# Autodesk Inventor assembly: ParticleLauncherwCollector
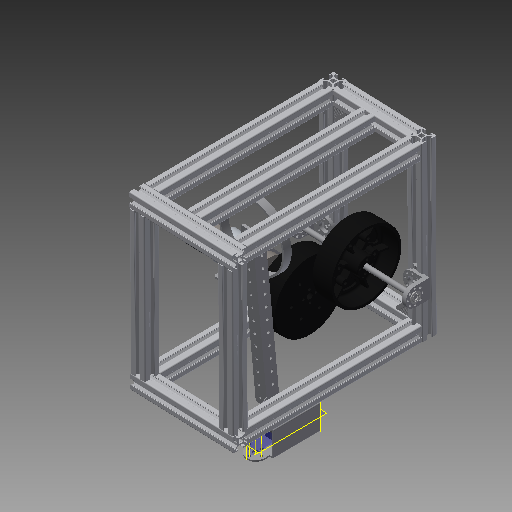
[picture p0: Inventor's stored thumbnail of the model, 512x512]
Saved by Autodesk Inventor 2017 (Build 210142000, 142)
## iProperties
Created: 2016-10-12
Part Number: ParticleLauncherwCollector
Document SubType Name: Assembly
Designer: Delta
Author: Delta
## Documents named in this file (20)
- C:\Robotics\CAD\2016-17_CAD\ParticleLauncher2.0.iam
- C:\Robotics\CAD\COTSParts\Actobotics\555 parts\555116.ipt
- C:\Robotics\CAD\COTSParts\Actobotics\am-3102NeveRest20 (1).ipt
- C:\Robotics\CAD\COTSParts\Actobotics\634 parts\634088.ipt
- C:\Robotics\CAD\COTSParts\Wheels\4in Wheel Intergreated Hub 8mm Rev2.ipt
- C:\Robotics\CAD\COTSParts\Bearings - AndyMark\Bearing 250 ID 500 OD flanged.ipt
- C:\Robotics\CAD\COTSParts\Actobotics\545 parts\545400.ipt
- C:\Robotics\CAD\COTSParts\Bosch Extrusion\6mm block nut M4.ipt
- C:\Robotics\CAD\COTSParts\Bosch Extrusion\Bosch 20x20 - 4.5 Part.Shoot.ipt
- C:\Robotics\CAD\COTSParts\Bosch Extrusion\Gusset 20x20 w screws.ipt
- C:\Robotics\CAD\COTSParts\Bosch Extrusion\Bosch 20x20 13 in.ipt
- C:\Robotics\CAD\COTSParts\Actobotics\585 parts\585422.ipt
- C:\Robotics\CAD\COTSParts\Bosch Extrusion\Bosch 20x20 9 real.ipt
- C:\Robotics\CAD\COTSParts\Bosch Extrusion\Bosch 20x20 7.675.ipt
- C:\Robotics\CAD\COTSParts\Bosch Extrusion\Bosch 20x20 5.5.ipt
- C:\Robotics\CAD\2016-17_CAD\popper.ipt
- C:\Robotics\CAD\COTSParts\Tetrix\Tetrix servo 180.ipt
- C:\Robotics\CAD\COTSParts\Tetrix\Tetrix angle 288mm.ipt
- C:\Robotics\CAD\COTSParts\Bosch Extrusion\6mm block nut M5.ipt
- C:\Robotics\CAD\COTSParts\Tetrix\ptp_tetrix_servoframe_bracket.ipt
## Components (39 placed, 19 different names)
1. 555116:1 — Insert:15, Insert:48, Insert:49
2. am-3102NeveRest20 (1):1 — Insert:15, Insert:34
3. 634088:1 — Mate:73, Mate:74, Flush:9, Mate:75
4. 4in Wheel Intergreated Hub 8mm Rev2:1 — Mate:75, Mate:76
5. 4in Wheel Intergreated Hub 8mm Rev2:2 — Insert:34
6. Bearing 250 ID 500 OD flanged:2 — Mate:69, Mate:70, Mate:74
7. Bearing 250 ID 500 OD flanged:3 — Mate:71, Mate:72, Mate:73
8. 545400:1 — Insert:42, Insert:43, Mate:71, Mate:72, Flush:10
9. 545400:2 — Insert:44, Insert:45, Mate:69, Mate:70, Flush:9
10. 6mm block nut M4:1 — Mate:91, Mate:92, Insert:47
11. 6mm block nut M4:2 — Mate:89, Mate:90, Insert:46
12. 6mm block nut M4:4 — Insert:43, Mate:62
13. 6mm block nut M4:5 — Insert:42, Mate:63, Mate:64
14. 6mm block nut M4:6 — Insert:44, Mate:67, Mate:68
15. 6mm block nut M4:7 — Mate:46, Mate:47, Insert:45, Mate:65, Mate:66
16. Bosch 20x20 - 4.5 Part.Shoot:1 — Mate:30, Mate:31, Mate:34, Mate:35, Mate:45, Flush:3, Flush:4, Flush:5, Flush:6, Mate:48
17. Gusset 20x20 w screws:1 — Mate:30, Mate:31, Mate:53
18. Gusset 20x20 w screws:2 — Mate:34, Mate:35, Mate:52
19. Bosch 20x20 13 in:1 — Flush:5, Flush:6, Mate:48, Mate:53, Mate:56, Mate:57, Mate:58, Flush:8, Mate:62, Mate:63, Mate:64, Flush:10, Mate:76, Mate:77, Flush:11, Flush:12, Mate:80, Flush:17, Flush:18, Mate:82, Flush:26
20. Bosch 20x20 13 in:2 — Mate:45, Flush:3, Flush:4, Mate:46, Mate:47, Mate:52, Mate:61, Mate:65, Mate:66, Mate:67, Mate:68, Mate:78, Flush:13, Flush:14, Mate:79, Flush:15, Flush:16
21. Bosch 20x20 - 4.5 Part.Shoot:2 — Mate:54, Mate:55, Mate:58, Flush:8, Mate:59, Mate:60, Mate:81, Flush:19
22. Gusset 20x20 w screws:3 — Mate:54, Mate:55, Mate:56, Mate:57
23. Gusset 20x20 w screws:4 — Mate:59, Mate:60, Mate:61
24. 585422:1 — Insert:46, Insert:47, Insert:48, Insert:49, Flush:26
25. Bosch 20x20 9 real:1 — Mate:79, Flush:15, Flush:16, Mate:86, Flush:21, Flush:27, Mate:99
26. Bosch 20x20 9 real:2 — Mate:77, Flush:11, Flush:12, Mate:83, Flush:20, Flush:22, Flush:23
27. Bosch 20x20 9 real:3 — Mate:78, Flush:13, Flush:14, Mate:85, Tangent:2
28. Bosch 20x20 9 real:4 — Mate:81, Flush:19, Mate:82, Mate:87, Tangent:1
29. Bosch 20x20 9 real:5 — Mate:80, Flush:17, Flush:18, Mate:84, Mate:88, Flush:25, Mate:89, Mate:90, Mate:91, Mate:92, Mate:94, Mate:95, Mate:97, Mate:98
30. Bosch 20x20 7.675:1 — Mate:85, Mate:86, Flush:21
31. Bosch 20x20 7.675:2 — Mate:83, Mate:84, Flush:20, Flush:24
32. Bosch 20x20 5.5:1 — Mate:88, Flush:24, Flush:25, Mate:96, Mate:100
33. Bosch 20x20 5.5:2 — Mate:87, Flush:22, Flush:23, Mate:93
34. popper:1 — Tangent:1, Mate:93, Tangent:2
35. Tetrix servo 180:1 — Insert:52, Insert:53, Mate:100
36. Tetrix angle 288mm:1 — Insert:52
37. 6mm block nut M5:1 — Mate:97, Mate:98
38. 6mm block nut M5:2 — Mate:94, Mate:95, Mate:96
39. ptp_tetrix_servoframe_bracket:1 — Flush:27, Mate:99, Insert:53
## Relationships (95: Mate 57, Flush 24, Insert 12, Tangent 2)
- Insert:15 (-9.525 mm): 555116:1 ↔ am-3102NeveRest20 (1):1
- Insert:34 (-10.16 mm): am-3102NeveRest20 (1):1 ↔ 4in Wheel Intergreated Hub 8mm Rev2:2
- Mate:30: Bosch 20x20 - 4.5 Part.Shoot:1 ↔ Gusset 20x20 w screws:1
- Mate:31: Bosch 20x20 - 4.5 Part.Shoot:1 ↔ Gusset 20x20 w screws:1
- Mate:34: Bosch 20x20 - 4.5 Part.Shoot:1 ↔ Gusset 20x20 w screws:2
- Mate:35: Bosch 20x20 - 4.5 Part.Shoot:1 ↔ Gusset 20x20 w screws:2
- Mate:45: Bosch 20x20 - 4.5 Part.Shoot:1 ↔ Bosch 20x20 13 in:2
- Flush:3: Bosch 20x20 - 4.5 Part.Shoot:1 ↔ Bosch 20x20 13 in:2
- Flush:4: Bosch 20x20 - 4.5 Part.Shoot:1 ↔ Bosch 20x20 13 in:2
- Mate:46: 6mm block nut M4:7 ↔ Bosch 20x20 13 in:2
- Mate:47: 6mm block nut M4:7 ↔ Bosch 20x20 13 in:2
- Flush:5: Bosch 20x20 - 4.5 Part.Shoot:1 ↔ Bosch 20x20 13 in:1
- Flush:6: Bosch 20x20 - 4.5 Part.Shoot:1 ↔ Bosch 20x20 13 in:1
- Mate:48: Bosch 20x20 - 4.5 Part.Shoot:1 ↔ Bosch 20x20 13 in:1
- Mate:52: Gusset 20x20 w screws:2 ↔ Bosch 20x20 13 in:2
- Mate:53: Gusset 20x20 w screws:1 ↔ Bosch 20x20 13 in:1
- Mate:54: Bosch 20x20 - 4.5 Part.Shoot:2 ↔ Gusset 20x20 w screws:3
- Mate:55: Bosch 20x20 - 4.5 Part.Shoot:2 ↔ Gusset 20x20 w screws:3
- Mate:56: Bosch 20x20 13 in:1 ↔ Gusset 20x20 w screws:3
- Mate:57: Bosch 20x20 13 in:1 ↔ Gusset 20x20 w screws:3
- Mate:58: Bosch 20x20 13 in:1 ↔ Bosch 20x20 - 4.5 Part.Shoot:2
- Flush:8: Bosch 20x20 13 in:1 ↔ Bosch 20x20 - 4.5 Part.Shoot:2
- Mate:59: Bosch 20x20 - 4.5 Part.Shoot:2 ↔ Gusset 20x20 w screws:4
- Mate:60: Bosch 20x20 - 4.5 Part.Shoot:2 ↔ Gusset 20x20 w screws:4
- Mate:61: Bosch 20x20 13 in:2 ↔ Gusset 20x20 w screws:4
- Insert:42: 545400:1 ↔ 6mm block nut M4:5
- Insert:43: 545400:1 ↔ 6mm block nut M4:4
- Mate:62: 6mm block nut M4:4 ↔ Bosch 20x20 13 in:1
- Mate:63: 6mm block nut M4:5 ↔ Bosch 20x20 13 in:1
- Mate:64: 6mm block nut M4:5 ↔ Bosch 20x20 13 in:1
- Insert:44: 545400:2 ↔ 6mm block nut M4:6
- Insert:45: 545400:2 ↔ 6mm block nut M4:7
- Mate:65: 6mm block nut M4:7 ↔ Bosch 20x20 13 in:2
- Mate:66: 6mm block nut M4:7 ↔ Bosch 20x20 13 in:2
- Mate:67: 6mm block nut M4:6 ↔ Bosch 20x20 13 in:2
- Mate:68: 6mm block nut M4:6 ↔ Bosch 20x20 13 in:2
- Mate:69: Bearing 250 ID 500 OD flanged:2 ↔ 545400:2
- Mate:70: Bearing 250 ID 500 OD flanged:2 ↔ 545400:2
- Mate:71: Bearing 250 ID 500 OD flanged:3 ↔ 545400:1
- Mate:72: Bearing 250 ID 500 OD flanged:3 ↔ 545400:1
- Mate:73: 634088:1 ↔ Bearing 250 ID 500 OD flanged:3
- Mate:74: 634088:1 ↔ Bearing 250 ID 500 OD flanged:2
- Flush:9: 634088:1 ↔ 545400:2
- Mate:75: 634088:1 ↔ 4in Wheel Intergreated Hub 8mm Rev2:1
- Flush:10 (55.88 mm): 545400:1 ↔ Bosch 20x20 13 in:1
- Mate:76 (37.1475 mm): 4in Wheel Intergreated Hub 8mm Rev2:1 ↔ Bosch 20x20 13 in:1
- Mate:77: Bosch 20x20 13 in:1 ↔ Bosch 20x20 9 real:2
- Flush:11: Bosch 20x20 13 in:1 ↔ Bosch 20x20 9 real:2
- Flush:12: Bosch 20x20 13 in:1 ↔ Bosch 20x20 9 real:2
- Mate:78: Bosch 20x20 13 in:2 ↔ Bosch 20x20 9 real:3
- Flush:13: Bosch 20x20 13 in:2 ↔ Bosch 20x20 9 real:3
- Flush:14: Bosch 20x20 13 in:2 ↔ Bosch 20x20 9 real:3
- Mate:79: Bosch 20x20 13 in:2 ↔ Bosch 20x20 9 real:1
- Flush:15: Bosch 20x20 13 in:2 ↔ Bosch 20x20 9 real:1
- Flush:16: Bosch 20x20 13 in:2 ↔ Bosch 20x20 9 real:1
- Mate:80: Bosch 20x20 13 in:1 ↔ Bosch 20x20 9 real:5
- Flush:17: Bosch 20x20 13 in:1 ↔ Bosch 20x20 9 real:5
- Flush:18: Bosch 20x20 13 in:1 ↔ Bosch 20x20 9 real:5
- Mate:81: Bosch 20x20 - 4.5 Part.Shoot:2 ↔ Bosch 20x20 9 real:4
- Flush:19: Bosch 20x20 - 4.5 Part.Shoot:2 ↔ Bosch 20x20 9 real:4
- Mate:82 (37.1475 mm): Bosch 20x20 13 in:1 ↔ Bosch 20x20 9 real:4
- Mate:83: Bosch 20x20 9 real:2 ↔ Bosch 20x20 7.675:2
- Mate:84: Bosch 20x20 9 real:5 ↔ Bosch 20x20 7.675:2
- Flush:20: Bosch 20x20 9 real:2 ↔ Bosch 20x20 7.675:2
- Mate:85: Bosch 20x20 9 real:3 ↔ Bosch 20x20 7.675:1
- Mate:86: Bosch 20x20 9 real:1 ↔ Bosch 20x20 7.675:1
- Flush:21: Bosch 20x20 9 real:1 ↔ Bosch 20x20 7.675:1
- Mate:87: Bosch 20x20 9 real:4 ↔ Bosch 20x20 5.5:2
- Flush:22: Bosch 20x20 9 real:2 ↔ Bosch 20x20 5.5:2
- Flush:23: Bosch 20x20 9 real:2 ↔ Bosch 20x20 5.5:2
- Mate:88: Bosch 20x20 9 real:5 ↔ Bosch 20x20 5.5:1
- Flush:24: Bosch 20x20 7.675:2 ↔ Bosch 20x20 5.5:1
- Flush:25: Bosch 20x20 9 real:5 ↔ Bosch 20x20 5.5:1
- Mate:89: 6mm block nut M4:2 ↔ Bosch 20x20 9 real:5
- Mate:90: 6mm block nut M4:2 ↔ Bosch 20x20 9 real:5
- Mate:91: 6mm block nut M4:1 ↔ Bosch 20x20 9 real:5
- Mate:92: 6mm block nut M4:1 ↔ Bosch 20x20 9 real:5
- Insert:46: 6mm block nut M4:2 ↔ 585422:1
- Insert:47: 6mm block nut M4:1 ↔ 585422:1
- Insert:48: 555116:1 ↔ 585422:1
- Insert:49: 555116:1 ↔ 585422:1
- Flush:26 (68.58 mm): Bosch 20x20 13 in:1 ↔ 585422:1
- Tangent:1: Bosch 20x20 9 real:4 ↔ popper:1
- Mate:93 (73.025 mm): Bosch 20x20 5.5:2 ↔ popper:1
- Tangent:2 (6.096 mm): Bosch 20x20 9 real:3 ↔ popper:1
- Mate:94: Bosch 20x20 9 real:5 ↔ 6mm block nut M5:2
- Mate:95: Bosch 20x20 9 real:5 ↔ 6mm block nut M5:2
- Mate:96 (40.64 mm): Bosch 20x20 5.5:1 ↔ 6mm block nut M5:2
- Mate:97: Bosch 20x20 9 real:5 ↔ 6mm block nut M5:1
- Mate:98: Bosch 20x20 9 real:5 ↔ 6mm block nut M5:1
- Insert:52: Tetrix servo 180:1 ↔ Tetrix angle 288mm:1
- Flush:27: Bosch 20x20 9 real:1 ↔ ptp_tetrix_servoframe_bracket:1
- Mate:99: Bosch 20x20 9 real:1 ↔ ptp_tetrix_servoframe_bracket:1
- Insert:53: Tetrix servo 180:1 ↔ ptp_tetrix_servoframe_bracket:1
- Mate:100 (44.45 mm): Bosch 20x20 5.5:1 ↔ Tetrix servo 180:1
